# Autodesk Inventor assembly: Lower skin assembly
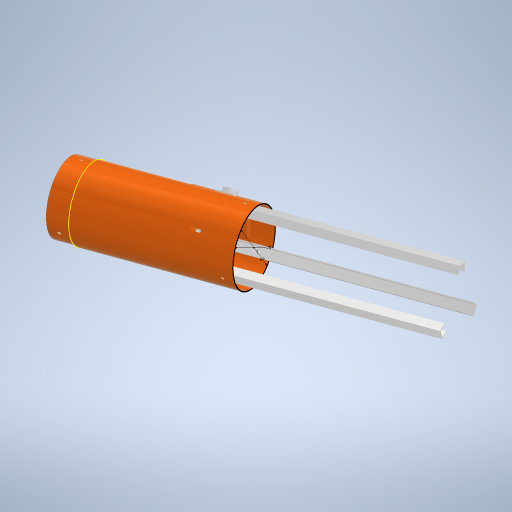
[picture p0: Inventor's stored thumbnail of the model, 512x512]
Saved by Autodesk Inventor 2024 (Build 280153000, 153)
## iProperties
Created: 2024-04-27
Part Number: Lower skin assembly
Document SubType Name: Assembly
Designer: auror
Author: auror
## Documents named in this file (6)
- C:\Users\auror\Documents\TU Delft\DARE\Git\Scrambler-2-CAD\Autodesk\Lower skin assembly.iam
- C:\Users\auror\Documents\TU Delft\DARE\Git\Scrambler-2-CAD\Autodesk\Electronics Door.ipt
- C:\Users\auror\Documents\TU Delft\DARE\Git\Scrambler-2-CAD\Autodesk\Lower skin.ipt
- C:\Users\auror\Documents\TU Delft\DARE\Git\Scrambler-2-CAD\Autodesk\Electronic Assembly.iam
- C:\Users\auror\Documents\TU Delft\DARE\Git\Scrambler-2-CAD\Autodesk\Button.ipt
- C:\Users\auror\Documents\TU Delft\DARE\Git\Scrambler-2-CAD\Autodesk\Stringer.ipt
## Components (8 placed, 5 different names)
1. Electronics Door:1 — Mate:24
2. Lower skin:1 — Mate:24, Mate:26, Mate:27, Mate:28, Mate:29, Mate:30, Angle:1, Angle:2, Mate:31, Mate:32, Mate:33, Mate:34, Mate:35, Mate:36, Mate:37, Mate:38, Mate:39, Mate:40
3. Electronic Assembly:1 [sub-assembly] — Mate:26, Mate:37
4. Button:1 — Mate:29, Mate:30, Angle:1
5. Button:2 — Mate:27, Mate:28, Angle:2
6. Stringer:1 — Mate:38, Mate:39, Mate:40
7. Stringer:2 — Mate:33, Mate:34, Mate:35
8. Stringer:3 — Mate:31, Mate:32, Mate:36
## Relationships (18: Mate 16, Angle 2)
- Mate:24: Electronics Door:1 ↔ Lower skin:1
- Mate:26: Lower skin:1 ↔ Electronic Assembly:1
- Mate:27: Lower skin:1 ↔ Button:2
- Mate:28: Lower skin:1 ↔ Button:2
- Mate:29: Lower skin:1 ↔ Button:1
- Mate:30: Lower skin:1 ↔ Button:1
- Angle:1 (0 deg): Lower skin:1 ↔ Button:1
- Angle:2 (0 deg): Lower skin:1 ↔ Button:2
- Mate:31: Lower skin:1 ↔ Stringer:3
- Mate:32: Lower skin:1 ↔ Stringer:3
- Mate:33: Lower skin:1 ↔ Stringer:2
- Mate:34: Lower skin:1 ↔ Stringer:2
- Mate:35 (-33 mm): Lower skin:1 ↔ Stringer:2
- Mate:36 (-33 mm): Lower skin:1 ↔ Stringer:3
- Mate:37: Lower skin:1 ↔ Electronic Assembly:1
- Mate:38: Lower skin:1 ↔ Stringer:1
- Mate:39: Lower skin:1 ↔ Stringer:1
- Mate:40 (-33 mm): Lower skin:1 ↔ Stringer:1
